# Autodesk Inventor assembly: Itemrahmen
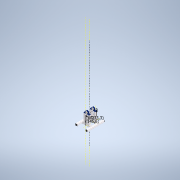
[picture p0: Inventor's stored thumbnail of the model, 180x180]
Saved by Autodesk Inventor 2022 (Build 260153000, 153)
## iProperties
Created: 2022-03-15
Part Number: Itemrahmen
Document SubType Name: Assembly
Designer: 123St
Gestell_Lager_Distanz: 145,600 mm
Gestell_Lager_Lochbreite: 87,000 mm
Author: 123St
## Documents named in this file (6)
- C:\Users\AEWALDER\Documents\Inventor\03_CurrentProjects\MasterThesis\PSM_V1_Rillenkugellager\Itemrahmen.iam
- C:\Users\AEWALDER\Documents\Inventor\03_CurrentProjects\MasterThesis\PSM_V1_Rillenkugellager\Item_500_Bodenfuss.ipt
- C:\Users\AEWALDER\Documents\Inventor\03_CurrentProjects\MasterThesis\PSM_V1_Rillenkugellager\Item_200_Bodenquerverbindung.ipt
- C:\Users\AEWALDER\Documents\Inventor\03_CurrentProjects\MasterThesis\PSM_V1_Rillenkugellager\Item_400_Streben.ipt
- C:\Users\AEWALDER\Documents\Inventor\03_CurrentProjects\MasterThesis\PSM_V1_Rillenkugellager\Maschinenbauteil\item_0049433_abdeckkappe_profil_st_8_40x40_details_3.ipt
- C:\Users\AEWALDER\Documents\Inventor\03_CurrentProjects\MasterThesis\PSM_V1_Rillenkugellager\Maschinenbauteil\snr_esp204_0.ipt
## Components (14 placed, 5 different names)
1. Item_500_Bodenfuss:1 — Fluchtend:1, Passend:1, Fluchtend:2, Passend:26, Passend:27, Symmetrie:1, Passend:45, Passend:46
2. Item_500_Bodenfuss:2 — Passend:2, Fluchtend:3, Fluchtend:4, Passend:3, Fluchtend:5, Fluchtend:6, Passend:24, Passend:25, Symmetrie:1, Passend:43, Passend:44
3. Item_200_Bodenquerverbindung:1 — Fluchtend:1, Passend:1, Fluchtend:2, Passend:2, Fluchtend:3, Fluchtend:4, Passend:4, Fluchtend:7, Passend:5, Fluchtend:8, Passend:42
4. Item_200_Bodenquerverbindung:2 — Passend:3, Fluchtend:5, Fluchtend:6, Passend:6, Fluchtend:9, Passend:7, Fluchtend:10
5. Item_400_Streben:1 — Passend:7, Fluchtend:10, Passend:9, Passend:13, Symmetrie:2
6. Item_400_Streben:2 — Passend:4, Fluchtend:7, Passend:8, Passend:14, Symmetrie:3
7. Item_400_Streben:3 — Passend:5, Fluchtend:8, Passend:8, Passend:15, Symmetrie:3, Passend:38, Passend:39
8. Item_400_Streben:4 — Passend:6, Fluchtend:9, Passend:9, Passend:12, Symmetrie:2, Passend:36, Passend:37
9. item_0049433_abdeckkappe_profil_st_8_40x40_details_3:1 — Passend:45, Passend:46
10. item_0049433_abdeckkappe_profil_st_8_40x40_details_3:2 — Passend:43, Passend:44
11. item_0049433_abdeckkappe_profil_st_8_40x40_details_3:3 — Passend:26, Passend:27
12. item_0049433_abdeckkappe_profil_st_8_40x40_details_3:4 — Passend:24, Passend:25
13. snr_esp204_0:1 — Passend:36, Passend:37
14. snr_esp204_0:2 — Passend:38, Passend:39
## Relationships (49: Mate 36, Flush 10, Symmetry 3)
- Fluchtend:1 [Flush]: Item_500_Bodenfuss:1 ↔ Item_200_Bodenquerverbindung:1
- Passend:1 [Mate]: Item_500_Bodenfuss:1 ↔ Item_200_Bodenquerverbindung:1
- Fluchtend:2 [Flush] (100 mm): Item_500_Bodenfuss:1 ↔ Item_200_Bodenquerverbindung:1
- Passend:2 [Mate]: Item_500_Bodenfuss:2 ↔ Item_200_Bodenquerverbindung:1
- Fluchtend:3 [Flush]: Item_500_Bodenfuss:2 ↔ Item_200_Bodenquerverbindung:1
- Fluchtend:4 [Flush] (100 mm): Item_500_Bodenfuss:2 ↔ Item_200_Bodenquerverbindung:1
- Passend:3 [Mate]: Item_500_Bodenfuss:2 ↔ Item_200_Bodenquerverbindung:2
- Fluchtend:5 [Flush]: Item_500_Bodenfuss:2 ↔ Item_200_Bodenquerverbindung:2
- Fluchtend:6 [Flush] (245.6 mm): Item_500_Bodenfuss:2 ↔ Item_200_Bodenquerverbindung:2
- Passend:4 [Mate]: Item_200_Bodenquerverbindung:1 ↔ Item_400_Streben:2
- Fluchtend:7 [Flush]: Item_200_Bodenquerverbindung:1 ↔ Item_400_Streben:2
- Passend:5 [Mate]: Item_200_Bodenquerverbindung:1 ↔ Item_400_Streben:3
- Fluchtend:8 [Flush]: Item_200_Bodenquerverbindung:1 ↔ Item_400_Streben:3
- Passend:6 [Mate]: Item_200_Bodenquerverbindung:2 ↔ Item_400_Streben:4
- Fluchtend:9 [Flush]: Item_200_Bodenquerverbindung:2 ↔ Item_400_Streben:4
- Passend:7 [Mate]: Item_200_Bodenquerverbindung:2 ↔ Item_400_Streben:1
- Fluchtend:10 [Flush]: Item_200_Bodenquerverbindung:2 ↔ Item_400_Streben:1
- Passend:8 [Mate] (47 mm): Item_400_Streben:2 ↔ Item_400_Streben:3
- Passend:9 [Mate] (47 mm): Item_400_Streben:1 ↔ Item_400_Streben:4
- Passend:12 [Mate]: Item_400_Streben:4
- Passend:13 [Mate]: Item_400_Streben:1
- Passend:14 [Mate]: Item_400_Streben:2
- Passend:15 [Mate]: Item_400_Streben:3
- Passend:16 [Mate]
- Passend:17 [Mate]
- Passend:18 [Mate]
- Passend:19 [Mate]
- Passend:20 [Mate]
- Passend:21 [Mate]
- Passend:24 [Mate]: Item_500_Bodenfuss:2 ↔ item_0049433_abdeckkappe_profil_st_8_40x40_details_3:4
- Passend:25 [Mate]: Item_500_Bodenfuss:2 ↔ item_0049433_abdeckkappe_profil_st_8_40x40_details_3:4
- Passend:26 [Mate]: Item_500_Bodenfuss:1 ↔ item_0049433_abdeckkappe_profil_st_8_40x40_details_3:3
- Passend:27 [Mate]: Item_500_Bodenfuss:1 ↔ item_0049433_abdeckkappe_profil_st_8_40x40_details_3:3
- Symmetrie:1: Item_500_Bodenfuss:1 ↔ Item_500_Bodenfuss:2
- Symmetrie:2: Item_400_Streben:1 ↔ Item_400_Streben:4
- Passend:32 [Mate]
- Symmetrie:3: Item_400_Streben:2 ↔ Item_400_Streben:3
- Passend:33 [Mate]
- Passend:36 [Mate]: Item_400_Streben:4 ↔ snr_esp204_0:1
- Passend:37 [Mate]: Item_400_Streben:4 ↔ snr_esp204_0:1
- Passend:38 [Mate]: Item_400_Streben:3 ↔ snr_esp204_0:2
- Passend:39 [Mate]: Item_400_Streben:3 ↔ snr_esp204_0:2
- Passend:40 [Mate]
- Passend:41 [Mate]
- Passend:42 [Mate]: Item_200_Bodenquerverbindung:1
- Passend:43 [Mate]: Item_500_Bodenfuss:2 ↔ item_0049433_abdeckkappe_profil_st_8_40x40_details_3:2
- Passend:44 [Mate]: Item_500_Bodenfuss:2 ↔ item_0049433_abdeckkappe_profil_st_8_40x40_details_3:2
- Passend:45 [Mate]: Item_500_Bodenfuss:1 ↔ item_0049433_abdeckkappe_profil_st_8_40x40_details_3:1
- Passend:46 [Mate]: Item_500_Bodenfuss:1 ↔ item_0049433_abdeckkappe_profil_st_8_40x40_details_3:1
## Named parameters: Gestell_Lager_Distanz = 145.6 mm, Gestell_Lager_Lochbreite = 87 mm, ItemWidth = 40 mm
